# Autodesk Inventor assembly: RodAssembly
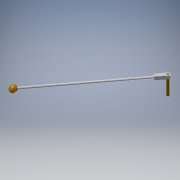
[picture p0: Inventor's stored thumbnail of the model, 180x180]
Saved by Autodesk Inventor 2016 (Build 200138000, 138)
## iProperties
Created: 2015-05-19
Part Number: RodAssembly
Document SubType Name: Assembly
Designer: Andy
Mass: 262 g
Surface Area: 191.877 cm^2
Volume: 47.4931 cm^3
Density: 5.51659 g/cm^3
Author: Andy
## Documents named in this file (4)
- C:\Users\jonathan\Documents\GitHub\Integrated-Tool-Suite\Inverted Pendulum\Inventor\Pendulum Assembly.iam
- C:\Users\jonathan\Documents\GitHub\Integrated-Tool-Suite\Inverted Pendulum\Inventor\Pendulum Rod.ipt
- C:\Users\jonathan\Documents\GitHub\Integrated-Tool-Suite\Inverted Pendulum\Inventor\Pendulum Axle.ipt
- C:\Users\jonathan\Documents\GitHub\Integrated-Tool-Suite\Inverted Pendulum\Inventor\Pendulum Brass Weight.ipt
## Components (3 placed, 3 different names)
1. Pendulum Rod:1 — Mate:5, Flush:1, Mate:6
2. Pendulum Axle:1 — Mate:5, Flush:1
3. Pendulum Brass Weight:1 — Mate:6
## Relationships (3: Mate 2, Flush 1)
- Mate:5: Pendulum Rod:1 ↔ Pendulum Axle:1
- Flush:1: Pendulum Rod:1 ↔ Pendulum Axle:1
- Mate:6: Pendulum Rod:1 ↔ Pendulum Brass Weight:1
